# Autodesk Inventor assembly: led
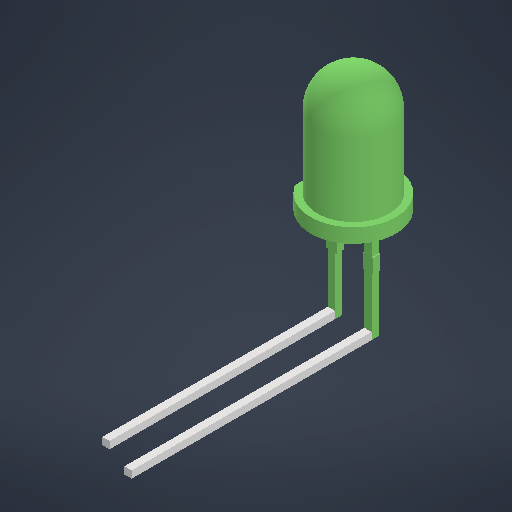
[picture p0: Inventor's stored thumbnail of the model, 512x512]
Saved by Autodesk Inventor 2025.2 (Build 292293000, 293)
## iProperties
Created: 2025-12-13
Part Number: led
Document SubType Name: Assembly
Designer: sam
Author: sam
## iProperties of the stored document WP7113ID_WP7113ID.ipt
Created: 2025-12-13
Part Number: WP7113ID_WP7113ID
Material: Generic
Document SubType Name: Modeling
Designer: sam
Density: 1 g/cm^3
Appearance: Default
Author: sam
Revision Number: ANY
## iProperties of the stored document WP7113ID.iam
Created: 2023-03-13
Part Number: WP7113ID
Description: STEP AP214
Document SubType Name: Assembly
Designer: sam
Sending System: SolidWorks 2021
Preprocessor: SwSTEP 2.0
Title: WP7113ID.STEP
Revision Number: ANY
## Documents named in this file (6)
- G:\projects\primary\regulated-irrigation-system\model\asm\pcb\led\led.iam
- **G:\projects\primary\regulated-irrigation-system\model\asm\pcb\led\led.iam*LocalDocs*xAaaaqxdaAaaaaaaaAaaaagetMf*WP7113ID.iam
- G:\projects\primary\regulated-irrigation-system\model\asm\pcb\led\led-wire-long.ipt
- G:\projects\primary\regulated-irrigation-system\model\asm\pcb\led\led-wire-short.ipt
- **G:\projects\primary\regulated-irrigation-system\model\asm\pcb\led\led.iam*LocalDocs*xAaaaqaaaAaaaaaaaAaaaqob5Dh*WP7113ID_WP7113ID.ipt
- G:\docs\kicad-libraries\WP7113ID\WP7113ID.step
## Components (3 placed, 3 different names)
1. WP7113ID:1 [sub-assembly] — Mate:1, Flush:1, Flush:2, Mate:2, Flush:3, Flush:4
2. led-wire-long:1 — Mate:1, Flush:1, Flush:2
3. led-wire-short:1 — Mate:2, Flush:3, Flush:4
## Relationships (6: Flush 4, Mate 2)
- Mate:1: WP7113ID:1 ↔ led-wire-long:1
- Flush:1: WP7113ID:1 ↔ led-wire-long:1
- Flush:2: WP7113ID:1 ↔ led-wire-long:1
- Mate:2: WP7113ID:1 ↔ led-wire-short:1
- Flush:3: WP7113ID:1 ↔ led-wire-short:1
- Flush:4: WP7113ID:1 ↔ led-wire-short:1
